# Autodesk Inventor assembly: caja
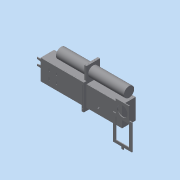
[picture p0: Inventor's stored thumbnail of the model, 180x180]
Saved by Autodesk Inventor 2015 (Build 190159000, 159)
## iProperties
Created: 2017-09-28
Part Number: caja
Document SubType Name: Assembly
Designer: Max
Author: Max
## Documents named in this file (12)
- \\Mac\Home\Dropbox\cosplay\caja\caja.iam
- \\Mac\Home\Dropbox\cosplay\caja\ladofuera.ipt
- \\Mac\Home\Dropbox\cosplay\caja\techo.ipt
- \\Mac\Home\Dropbox\cosplay\caja\ladodentro.ipt
- \\Mac\Home\Dropbox\cosplay\caja\piso.ipt
- \\Mac\Home\Dropbox\cosplay\caja\tapadelante.ipt
- \\Mac\Home\Dropbox\cosplay\caja\tapatras.ipt
- \\Mac\Home\Dropbox\cosplay\caja\sables.ipt
- \\Mac\Home\Dropbox\cosplay\caja\anillo.ipt
- \\Mac\Home\Dropbox\cosplay\caja\gas.ipt
- \\Mac\Home\Dropbox\cosplay\caja\anillo2.ipt
- \\Mac\Home\Dropbox\cosplay\caja\anillo3.ipt
## Components (13 placed, 11 different names)
1. ladofuera:1 — Flush:1, Mate:1, Flush:2, Mate:3, Flush:6
2. techo:1 — Flush:1, Mate:1, Flush:2, Flush:3, Mate:2, Flush:4, Mate:7, Flush:9
3. ladodentro:1 — Flush:3, Mate:2, Flush:4, Flush:5, Mate:12
4. piso:1 — Flush:5, Mate:3, Flush:6, Flush:7, Flush:8, Mate:4, Mate:5, Mate:6, Mate:11
5. tapadelante:1 — Flush:7, Flush:8, Mate:4, Mate:5, Mate:8, Mate:9, Mate:10
6. tapatras:1 — Mate:6, Mate:7, Flush:9
7. sables:1 — Mate:8, Mate:9, Mate:10
8. anillo:1 — Mate:11, Mate:12, Cylindrical:1, Mate:13, Flush:10, Flush:11, Flush:13, Flush:14, Flush:15, Mate:15
9. gas:1 — Cylindrical:1
10. anillo:2 — Mate:14, Flush:12, Flush:13
11. anillo:3
12. anillo2:1 — Mate:13, Flush:10, Flush:11, Mate:14, Flush:12
13. anillo3:1 — Flush:14, Flush:15, Mate:15
## Relationships (31: Flush 15, Mate 15, CylindricalJoint 1)
- Flush:1: ladofuera:1 ↔ techo:1
- Mate:1: ladofuera:1 ↔ techo:1
- Flush:2: ladofuera:1 ↔ techo:1
- Flush:3: techo:1 ↔ ladodentro:1
- Mate:2: techo:1 ↔ ladodentro:1
- Flush:4: techo:1 ↔ ladodentro:1
- Flush:5: ladodentro:1 ↔ piso:1
- Mate:3: ladofuera:1 ↔ piso:1
- Flush:6: ladofuera:1 ↔ piso:1
- Flush:7: piso:1 ↔ tapadelante:1
- Flush:8: piso:1 ↔ tapadelante:1
- Mate:4: piso:1 ↔ tapadelante:1
- Mate:5: piso:1 ↔ tapadelante:1
- Mate:6: piso:1 ↔ tapatras:1
- Mate:7: techo:1 ↔ tapatras:1
- Flush:9: techo:1 ↔ tapatras:1
- Mate:8: tapadelante:1 ↔ sables:1
- Mate:9: tapadelante:1 ↔ sables:1
- Mate:10: tapadelante:1 ↔ sables:1
- Mate:11: piso:1 ↔ anillo:1
- Mate:12: ladodentro:1 ↔ anillo:1
- Cylindrical:1: anillo:1 ↔ gas:1
- Mate:13: anillo:1 ↔ anillo2:1
- Flush:10: anillo:1 ↔ anillo2:1
- Flush:11: anillo:1 ↔ anillo2:1
- Mate:14: anillo:2 ↔ anillo2:1
- Flush:12: anillo:2 ↔ anillo2:1
- Flush:13: anillo:1 ↔ anillo:2
- Flush:14: anillo:1 ↔ anillo3:1
- Flush:15: anillo:1 ↔ anillo3:1
- Mate:15: anillo:1 ↔ anillo3:1
